# Autodesk Inventor assembly: concept
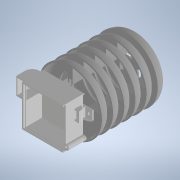
[picture p0: Inventor's stored thumbnail of the model, 180x180]
Saved by Autodesk Inventor 2020.3 (Build 243373000, 373)
## iProperties
Created: 2021-03-07
Part Number: concept
Document SubType Name: Assembly
Designer: sitar
Author: sitar
## Documents named in this file (5)
- C:\Users\sitar\GitHub\homeWeatherStation\cases\Inventor_2020\concept.iam
- C:\Users\sitar\GitHub\homeWeatherStation\cases\Inventor_2020\rib.ipt
- C:\Users\sitar\GitHub\homeWeatherStation\cases\Inventor_2020\holder.ipt
- C:\Users\sitar\GitHub\homeWeatherStation\cases\Inventor_2020\top_rib.ipt
- C:\Users\sitar\GitHub\homeWeatherStation\cases\Inventor_2020\PMS3003.ipt
## Components (8 placed, 4 different names)
1. rib:1 — Sztywne:1, Obrotowe:1
2. rib:2 — Sztywne:1, Sztywne:2
3. rib:3 — Obrotowe:2, Obrotowe:3
4. rib:4 — Obrotowe:1, Obrotowe:2
5. rib:5 — Sztywne:2, Sztywne:3
6. holder:1 — Obrotowe:3, Sztywne:4
7. top_rib:1 — Sztywne:3
8. PMS3003:1 — Sztywne:4
## Relationships (7: WeldJoint 4, RevoluteJoint 3)
- Sztywne:1 [WeldJoint]: rib:1 ↔ rib:2
- Obrotowe:1 [RevoluteJoint]: rib:1 ↔ rib:4
- Obrotowe:2 [RevoluteJoint]: rib:3 ↔ rib:4
- Sztywne:2 [WeldJoint]: rib:2 ↔ rib:5
- Obrotowe:3 [RevoluteJoint]: rib:3 ↔ holder:1
- Sztywne:3 [WeldJoint]: rib:5 ↔ top_rib:1
- Sztywne:4 [WeldJoint]: holder:1 ↔ PMS3003:1
